# Autodesk Inventor assembly: NewChassis
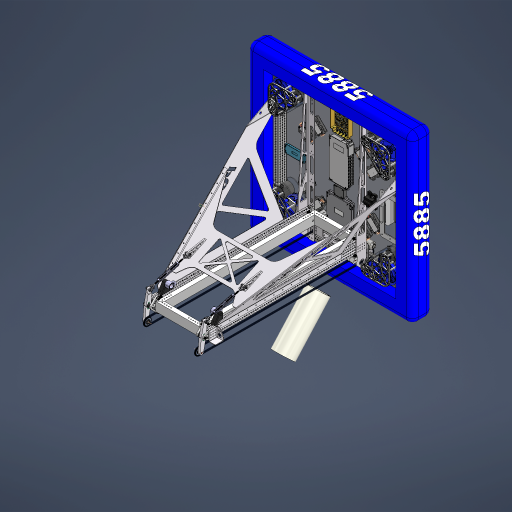
[picture p0: Inventor's stored thumbnail of the model, 512x512]
Saved by Autodesk Inventor 2024.3 (Build 283343000, 343)
## iProperties
ILogicPurgeVersion: 0.0.0.0
OnSaveVersion: 3.5.0.0
OnSaveAssembly: COREAutomationManager
Created: 2025-01-13
Part Number: NewChassis
Document SubType Name: Assembly
Designer: Marcus Tannini
Mfg Approved By: John.Thibert
Mass: 47914.5 g
Surface Area: 101218 cm^2
Volume: 49061.3 cm^3
Density: 0.976625 g/cm^3
ModelCat: Uncategorized
CN_MASS: 47.91
Author: Marcus Tannini
## Documents named in this file (44)
- \\clfs\homes\john.thibert\robot-test\#Poseidon 2025.iam
- \\clfs\homes\john.thibert\robot-test\ASSY,MK4i,Swerve_Module_INV.iam
- \\clfs\homes\john.thibert\robot-test\MAXTube-2x1-Holes.ipt
- \\clfs\homes\john.thibert\robot-test\BellyPanTop.ipt
- \\clfs\homes\john.thibert\robot-test\BellyPanBot.ipt
- \\clfs\homes\john.thibert\robot-test\BATTERY,12V.ipt
- \\clfs\homes\john.thibert\robot-test\CONTROLS,MAIN_BREAKER.ipt
- \\clfs\homes\john.thibert\robot-test\CONTROLS,MOTOR,NEO,550.ipt
- \\clfs\homes\john.thibert\robot-test\CONTROLS,PDH.ipt
- \\clfs\homes\john.thibert\robot-test\CONTROLS,PH.ipt
- \\clfs\homes\john.thibert\robot-test\CONTROLS,ROBO_RIO.ipt
- \\clfs\homes\john.thibert\robot-test\CONTROLS,SPARK_MAX.ipt
- \\clfs\homes\john.thibert\robot-test\CONTROLS,VRM.ipt
- \\clfs\homes\john.thibert\robot-test\COVER,SPARKMAX.ipt
- \\clfs\homes\john.thibert\robot-test\ModifiedCase(IncludesPatterning).iam
- \\clfs\homes\john.thibert\robot-test\PLATE,MOUNT,BATTERY,TOP.ipt
- \\clfs\homes\john.thibert\robot-test\PLATE,MOUNT,BATTERY,BOT.ipt
- \\clfs\homes\john.thibert\robot-test\MOUNT,STRAP,BATTERY.ipt
- \\clfs\homes\john.thibert\robot-test\SPACER,SPROCKET,IDLER,ELEVATOR.ipt
- \\clfs\homes\john.thibert\robot-test\22.ipt
- \\clfs\homes\john.thibert\robot-test\PLATE,MOUNT,DRIVE,ELEVATOR.ipt
- \\clfs\homes\john.thibert\robot-test\PLATE,BEARING,DRIVE,ELEVATOR.ipt
- \\clfs\homes\john.thibert\robot-test\PURCHASED,HEX_BEARING.ipt
- \\clfs\homes\john.thibert\robot-test\SHAFT,HEX,0.500in,DRIVE,ELEVATOR.ipt
- \\clfs\homes\john.thibert\robot-test\PLATE,SIDE,BRACE,RIGHT,ELEVATOR.ipt
- \\clfs\homes\john.thibert\robot-test\PLATE,SIDE,BRACE,LEFT,ELEVATOR.ipt
- \\clfs\homes\john.thibert\robot-test\PLATE,TURNBUCKLE,TENSIONER,CHAIN.ipt
- \\clfs\homes\john.thibert\robot-test\PLATE,BRACE,HORISONTAL,TOP,ELEVATOR.ipt
- \\clfs\homes\john.thibert\robot-test\TURNBUCKLE,0.25IN_CLEVIS.iam
- \\clfs\homes\john.thibert\robot-test\STAGE1,ELEVATOR.iam
- \\clfs\homes\john.thibert\robot-test\ASSY,MAIN,ELEVATOR.iam
- \\clfs\homes\john.thibert\robot-test\ANGLE,MOUNT,ELEVATOR.ipt
- \\clfs\homes\john.thibert\robot-test\ANGLE,MOUNT,ELEVATOR,MIRR.ipt
- \\clfs\homes\john.thibert\robot-test\FABRIC,BUMPERS.ipt
- \\clfs\homes\john.thibert\robot-test\9293K119_Constant-Force Spring.ipt
- \\clfs\homes\john.thibert\robot-test\MOUNT,SPRING,ELEVATOR.ipt
- \\clfs\homes\john.thibert\robot-test\MOUNT,SPRING,ELEVATOR,MIRR.ipt
- \\clfs\homes\john.thibert\robot-test\VersaPlanetary v2 Dual Stage 10_1 with RS 550 (1).iam
- \\clfs\homes\john.thibert\robot-test\60355K336_Ball Bearing.ipt
- \\clfs\homes\john.thibert\robot-test\91259A171_Alloy Steel Shoulder Screw.ipt
- \\clfs\homes\john.thibert\robot-test\BEARING,MOUNT,SIDE,ELEVATOR.ipt
- \\clfs\homes\john.thibert\robot-test\MOUNT,CABLE_TRACK,ELEVATOR.ipt
- \\clfs\homes\john.thibert\robot-test\CORAL.ipt
- \\clfs\homes\john.thibert\robot-test\BEARING,MOUNT,SIDE,ELEVATOR,MIRR.ipt
## Components (75 placed, 44 different names)
1. FABRIC,BUMPERS.ipt:1 — Flush:323, Mate:335, Mate:336
2. CORAL:1
3. BellyPanBot.ipt:1 — Mate:66, Mate:353, Mate:354
4. BellyPanTop.ipt:1 — Mate:62, Mate:63, Mate:65, Mate:70, Mate:71, Mate:82, Mate:84, Insert:7, Insert:8, Insert:9, Insert:10, Insert:11, Insert:12, Insert:13, Insert:14, Insert:15, Insert:16, Insert:17, Insert:18, Insert:19, Insert:20, Insert:21, Insert:22, Mate:111, Mate:113, Mate:114, Mate:116, Mate:117, Mate:118, Mate:119, Mate:121, Mate:122, Mate:123, Mate:124, Mate:125, Mate:126, Mate:127, Mate:130, Insert:23, Insert:24, Mate:223, Mate:308, Mate:320, Mate:349, Mate:350
5. MAXTube-2x1-Holes.ipt:1 — Mate:1, Mate:2, Mate:3, Mate:4, Mate:5, Mate:15, Mate:115, Mate:272
6. MAXTube-2x1-Holes.ipt:2 — Mate:6, Mate:7, Mate:8, Mate:9, Mate:10, Mate:11, Mate:62, Mate:309, Mate:310
7. MAXTube-2x1-Holes.ipt:3 — Mate:19, Mate:20, Mate:21, Mate:66, Mate:114, Mate:312, Mate:313, Mate:336
8. MAXTube-2x1-Holes.ipt:4 — Mate:12, Mate:13, Mate:14, Mate:16, Mate:17, Mate:18, Mate:29, Mate:63, Mate:271, Mate:353, Mate:354
9. MOUNT,STRAP,BATTERY.ipt:1 — Mate:357, Mate:358, Mate:359
10. PLATE,MOUNT,BATTERY,BOT.ipt:1 — Mate:320, Mate:321, Mate:351, Mate:352
11. PLATE,MOUNT,BATTERY,TOP.ipt:1 — Mate:127, Mate:349, Mate:350, Mate:351, Mate:352, Mate:356, Mate:357, Mate:358, Mate:359
12. BATTERY,12V.ipt:1 — Mate:321, Mate:356
13. CONTROLS,MAIN_BREAKER.ipt:1 — Mate:82, Mate:111, Mate:116
14. CONTROLS,MOTOR,NEO,550.ipt:1
15. CONTROLS,PDH.ipt:1 — Mate:113, Mate:117, Mate:118, Mate:119
16. CONTROLS,PH.ipt:1 — Insert:23, Insert:24
17. CONTROLS,ROBO_RIO.ipt:1 — Mate:124, Mate:125, Mate:126
18. CONTROLS,SPARK_MAX.ipt:1 — Mate:84, Mate:85, Mate:86, Mate:87
19. CONTROLS,VRM.ipt:1 — Mate:121, Mate:122, Mate:123
20. ModifiedCase(IncludesPatterning).iam:1 [sub-assembly] — Mate:130
21. 22.ipt:1 — Mate:227, Angle:6
22. 22.ipt:2 — Mate:233, Angle:4, Flush:14
23. 60355K336_Ball Bearing:1 — Mate:529, Mate:530, Mate:546
24. 60355K336_Ball Bearing:2 — Insert:51, Mate:545
25. 91259A171_Alloy Steel Shoulder Screw:1 — Mate:546
26. 91259A171_Alloy Steel Shoulder Screw:2 — Mate:545
27. 9293K119_Constant-Force Spring:1 — Mate:364, Mate:365
28. 9293K119_Constant-Force Spring:2 — Mate:370, Mate:371
29. ANGLE,MOUNT,ELEVATOR,MIRR.ipt:1 — Mate:308, Mate:309, Mate:310, Mate:311, Mate:312, Mate:313, Mate:314, Mate:315, Flush:329
30. ANGLE,MOUNT,ELEVATOR.ipt:1 — Mate:65, Mate:70, Mate:71, Mate:161, Mate:162, Mate:224, STAGE1 LOWER LIMIT, STAGE1 MIN
31. ASSY,MAIN,ELEVATOR.iam:1 [sub-assembly] — Mate:161, Mate:162, Flush:19, Mate:297, STAGE1 UPPER LIMIT, STAGE1 MAX, Mate:311, Mate:314, Mate:315, Mate:363, Mate:362, Mate:366, Mate:367, Mate:368, Mate:369, Mate:535, Mate:534, Mate:536
32. BEARING,MOUNT,SIDE,ELEVATOR,MIRR:1 — Mate:542, Mate:543, Mate:544, Insert:51
33. BEARING,MOUNT,SIDE,ELEVATOR:1 — Flush:330, Mate:528, Mate:529, Mate:530, Mate:531
34. CONTROLS,MOTOR,NEO,550:3
35. CONTROLS,MOTOR,NEO,550:4
36. MOUNT,CABLE_TRACK,ELEVATOR:1 — Mate:535, Mate:534, Mate:536
37. MOUNT,SPRING,ELEVATOR,MIRR:1 — Mate:367, Mate:368, Mate:369, Mate:370, Mate:371
38. MOUNT,SPRING,ELEVATOR:1 — Mate:363, Mate:362, Mate:364, Mate:365, Mate:366
39. PLATE,BEARING,DRIVE,ELEVATOR.ipt:1 — Mate:226, Mate:227, Mate:228, Mate:229, Insert:50
40. PLATE,BEARING,DRIVE,ELEVATOR.ipt:2 — Mate:230, Mate:231, Mate:232, Insert:49, Mate:233, Mate:234
41. PLATE,BRACE,HORISONTAL,TOP,ELEVATOR.ipt:1 — Mate:285, Mate:286, Mate:289, Mate:290, Mate:291, Mate:295, Mate:296
42. PLATE,MOUNT,DRIVE,ELEVATOR.ipt:1 — Mate:223, Mate:224, Mate:226, Mate:228, Mate:229, Mate:230, Mate:231, Mate:232, Flush:329, Mate:469, Mate:470, Mate:471, Mate:472, Mate:473, Mate:474
43. PLATE,SIDE,BRACE,LEFT,ELEVATOR.ipt:1 — Mate:271, Mate:289, Mate:290, Mate:291, Mate:335
44. PLATE,SIDE,BRACE,RIGHT,ELEVATOR.ipt:1 — Mate:272
45. PLATE,TURNBUCKLE,TENSIONER,CHAIN.ipt:1 — Mate:285, Mate:296
46. PLATE,TURNBUCKLE,TENSIONER,CHAIN.ipt:2 — Mate:286, Mate:295
47. PURCHASED,HEX_BEARING.ipt:1 — Insert:49, Angle:5
48. PURCHASED,HEX_BEARING.ipt:2 — Insert:50, Angle:7
49. SHAFT,HEX,0.500in,DRIVE,ELEVATOR.ipt:1 — Mate:234, Angle:4, Angle:5, Angle:6, Angle:7, Flush:14
50. SPACER,SPROCKET,IDLER,ELEVATOR.ipt:1
51. SPACER,SPROCKET,IDLER,ELEVATOR.ipt:2
52. STAGE1,ELEVATOR.iam:1 [sub-assembly] — Flush:19, Mate:297, STAGE1 LOWER LIMIT, STAGE1 UPPER LIMIT, STAGE1 MIN, STAGE1 MAX, Flush:330, Mate:528, Mate:531, Mate:542, Mate:543, Mate:544
53. TURNBUCKLE,0.25IN_CLEVIS.iam:1 [sub-assembly]
54. TURNBUCKLE,0.25IN_CLEVIS.iam:2 [sub-assembly]
55. VersaPlanetary v2 Dual Stage 10_1 with RS 550 (1):1 [sub-assembly] — Mate:472, Mate:473, Mate:474
56. VersaPlanetary v2 Dual Stage 10_1 with RS 550 (1):2 [sub-assembly] — Mate:469, Mate:470, Mate:471
57. ASSY,MK4i,Swerve_Module_INV.iam:1 [sub-assembly] — Mate:1, Mate:2, Mate:15
58. ASSY,MK4i,Swerve_Module_INV.iam:2 [sub-assembly] — Mate:3, Mate:4, Mate:5, Mate:6, Mate:7, Mate:8
59. ASSY,MK4i,Swerve_Module_INV.iam:3 [sub-assembly] — Mate:9, Mate:10, Mate:11, Mate:12, Mate:13, Mate:14
60. ASSY,MK4i,Swerve_Module_INV.iam:4 [sub-assembly] — Mate:16, Mate:17, Mate:18, Mate:19, Mate:20, Mate:21, Mate:67
61. CONTROLS,SPARK_MAX.ipt:2
62. CONTROLS,SPARK_MAX.ipt:3
63. CONTROLS,SPARK_MAX.ipt:4
64. CONTROLS,SPARK_MAX.ipt:5
65. CONTROLS,SPARK_MAX.ipt:6
66. CONTROLS,SPARK_MAX.ipt:7
67. CONTROLS,SPARK_MAX.ipt:8
68. COVER,SPARKMAX.ipt:1 — Mate:85, Mate:86, Mate:87, Insert:7, Insert:8
69. COVER,SPARKMAX.ipt:2 — Insert:9, Insert:10
70. COVER,SPARKMAX.ipt:3 — Insert:11, Insert:12
71. COVER,SPARKMAX.ipt:4 — Insert:13, Insert:14
72. COVER,SPARKMAX.ipt:5 — Insert:17, Insert:18
73. COVER,SPARKMAX.ipt:6 — Insert:15, Insert:16
74. COVER,SPARKMAX.ipt:7 — Insert:21, Insert:22
75. COVER,SPARKMAX.ipt:8 — Insert:19, Insert:20
## Relationships (203: Mate 167, Insert 25, Flush 7, Angle 4)
- Mate:1: MAXTube-2x1-Holes.ipt:1 ↔ ASSY,MK4i,Swerve_Module_INV.iam:1
- Mate:2: MAXTube-2x1-Holes.ipt:1 ↔ ASSY,MK4i,Swerve_Module_INV.iam:1
- Mate:3: MAXTube-2x1-Holes.ipt:1 ↔ ASSY,MK4i,Swerve_Module_INV.iam:2
- Mate:4: MAXTube-2x1-Holes.ipt:1 ↔ ASSY,MK4i,Swerve_Module_INV.iam:2
- Mate:5: MAXTube-2x1-Holes.ipt:1 ↔ ASSY,MK4i,Swerve_Module_INV.iam:2
- Mate:6: MAXTube-2x1-Holes.ipt:2 ↔ ASSY,MK4i,Swerve_Module_INV.iam:2
- Mate:7: MAXTube-2x1-Holes.ipt:2 ↔ ASSY,MK4i,Swerve_Module_INV.iam:2
- Mate:8: MAXTube-2x1-Holes.ipt:2 ↔ ASSY,MK4i,Swerve_Module_INV.iam:2
- Mate:9: MAXTube-2x1-Holes.ipt:2 ↔ ASSY,MK4i,Swerve_Module_INV.iam:3
- Mate:10: MAXTube-2x1-Holes.ipt:2 ↔ ASSY,MK4i,Swerve_Module_INV.iam:3
- Mate:11: MAXTube-2x1-Holes.ipt:2 ↔ ASSY,MK4i,Swerve_Module_INV.iam:3
- Mate:12: MAXTube-2x1-Holes.ipt:4 ↔ ASSY,MK4i,Swerve_Module_INV.iam:3
- Mate:13: MAXTube-2x1-Holes.ipt:4 ↔ ASSY,MK4i,Swerve_Module_INV.iam:3
- Mate:14: MAXTube-2x1-Holes.ipt:4 ↔ ASSY,MK4i,Swerve_Module_INV.iam:3
- Mate:15: MAXTube-2x1-Holes.ipt:1 ↔ ASSY,MK4i,Swerve_Module_INV.iam:1
- Mate:16: MAXTube-2x1-Holes.ipt:4 ↔ ASSY,MK4i,Swerve_Module_INV.iam:4
- Mate:17: MAXTube-2x1-Holes.ipt:4 ↔ ASSY,MK4i,Swerve_Module_INV.iam:4
- Mate:18: MAXTube-2x1-Holes.ipt:4 ↔ ASSY,MK4i,Swerve_Module_INV.iam:4
- Mate:19: MAXTube-2x1-Holes.ipt:3 ↔ ASSY,MK4i,Swerve_Module_INV.iam:4
- Mate:20: MAXTube-2x1-Holes.ipt:3 ↔ ASSY,MK4i,Swerve_Module_INV.iam:4
- Mate:21: MAXTube-2x1-Holes.ipt:3 ↔ ASSY,MK4i,Swerve_Module_INV.iam:4
- Mate:29 (-6.35 mm): MAXTube-2x1-Holes.ipt:4
- Mate:62: BellyPanTop.ipt:1 ↔ MAXTube-2x1-Holes.ipt:2
- Mate:63: BellyPanTop.ipt:1 ↔ MAXTube-2x1-Holes.ipt:4
- Mate:65: BellyPanTop.ipt:1 ↔ ANGLE,MOUNT,ELEVATOR.ipt:1
- Mate:66: BellyPanBot.ipt:1 ↔ MAXTube-2x1-Holes.ipt:3
- Mate:67 (35.56 mm): ASSY,MK4i,Swerve_Module_INV.iam:4
- Mate:70: BellyPanTop.ipt:1 ↔ ANGLE,MOUNT,ELEVATOR.ipt:1
- Mate:71: BellyPanTop.ipt:1 ↔ ANGLE,MOUNT,ELEVATOR.ipt:1
- Mate:321: PLATE,MOUNT,BATTERY,BOT.ipt:1 ↔ BATTERY,12V.ipt:1
- Mate:82: BellyPanTop.ipt:1 ↔ CONTROLS,MAIN_BREAKER.ipt:1
- Mate:84: BellyPanTop.ipt:1 ↔ CONTROLS,SPARK_MAX.ipt:1
- Mate:85: CONTROLS,SPARK_MAX.ipt:1 ↔ COVER,SPARKMAX.ipt:1
- Mate:86: CONTROLS,SPARK_MAX.ipt:1 ↔ COVER,SPARKMAX.ipt:1
- Mate:87: CONTROLS,SPARK_MAX.ipt:1 ↔ COVER,SPARKMAX.ipt:1
- Insert:7: BellyPanTop.ipt:1 ↔ COVER,SPARKMAX.ipt:1
- Insert:8: BellyPanTop.ipt:1 ↔ COVER,SPARKMAX.ipt:1
- [Mate]: CONTROLS,SPARK_MAX.ipt:2 ↔ COVER,SPARKMAX.ipt:2
- [Mate]: CONTROLS,SPARK_MAX.ipt:2 ↔ COVER,SPARKMAX.ipt:2
- [Mate]: CONTROLS,SPARK_MAX.ipt:2 ↔ COVER,SPARKMAX.ipt:2
- [Mate]: CONTROLS,SPARK_MAX.ipt:3 ↔ COVER,SPARKMAX.ipt:3
- [Mate]: CONTROLS,SPARK_MAX.ipt:3 ↔ COVER,SPARKMAX.ipt:3
- [Mate]: CONTROLS,SPARK_MAX.ipt:3 ↔ COVER,SPARKMAX.ipt:3
- [Mate]: CONTROLS,SPARK_MAX.ipt:4 ↔ COVER,SPARKMAX.ipt:4
- [Mate]: CONTROLS,SPARK_MAX.ipt:4 ↔ COVER,SPARKMAX.ipt:4
- [Mate]: CONTROLS,SPARK_MAX.ipt:4 ↔ COVER,SPARKMAX.ipt:4
- [Mate]: CONTROLS,SPARK_MAX.ipt:5 ↔ COVER,SPARKMAX.ipt:5
- [Mate]: CONTROLS,SPARK_MAX.ipt:5 ↔ COVER,SPARKMAX.ipt:5
- [Mate]: CONTROLS,SPARK_MAX.ipt:5 ↔ COVER,SPARKMAX.ipt:5
- [Mate]: CONTROLS,SPARK_MAX.ipt:6 ↔ COVER,SPARKMAX.ipt:6
- [Mate]: CONTROLS,SPARK_MAX.ipt:6 ↔ COVER,SPARKMAX.ipt:6
- [Mate]: CONTROLS,SPARK_MAX.ipt:6 ↔ COVER,SPARKMAX.ipt:6
- [Mate]: CONTROLS,SPARK_MAX.ipt:7 ↔ COVER,SPARKMAX.ipt:7
- [Mate]: CONTROLS,SPARK_MAX.ipt:7 ↔ COVER,SPARKMAX.ipt:7
- [Mate]: CONTROLS,SPARK_MAX.ipt:7 ↔ COVER,SPARKMAX.ipt:7
- [Mate]: CONTROLS,SPARK_MAX.ipt:8 ↔ COVER,SPARKMAX.ipt:8
- [Mate]: CONTROLS,SPARK_MAX.ipt:8 ↔ COVER,SPARKMAX.ipt:8
- [Mate]: CONTROLS,SPARK_MAX.ipt:8 ↔ COVER,SPARKMAX.ipt:8
- Insert:9: BellyPanTop.ipt:1 ↔ COVER,SPARKMAX.ipt:2
- Insert:10: BellyPanTop.ipt:1 ↔ COVER,SPARKMAX.ipt:2
- Insert:11: BellyPanTop.ipt:1 ↔ COVER,SPARKMAX.ipt:3
- Insert:12: BellyPanTop.ipt:1 ↔ COVER,SPARKMAX.ipt:3
- Insert:13: BellyPanTop.ipt:1 ↔ COVER,SPARKMAX.ipt:4
- Insert:14: BellyPanTop.ipt:1 ↔ COVER,SPARKMAX.ipt:4
- Insert:15: BellyPanTop.ipt:1 ↔ COVER,SPARKMAX.ipt:6
- Insert:16: BellyPanTop.ipt:1 ↔ COVER,SPARKMAX.ipt:6
- Insert:17: BellyPanTop.ipt:1 ↔ COVER,SPARKMAX.ipt:5
- Insert:18: BellyPanTop.ipt:1 ↔ COVER,SPARKMAX.ipt:5
- Insert:19: BellyPanTop.ipt:1 ↔ COVER,SPARKMAX.ipt:8
- Insert:20: BellyPanTop.ipt:1 ↔ COVER,SPARKMAX.ipt:8
- Insert:21: BellyPanTop.ipt:1 ↔ COVER,SPARKMAX.ipt:7
- Insert:22: BellyPanTop.ipt:1 ↔ COVER,SPARKMAX.ipt:7
- Mate:111: BellyPanTop.ipt:1 ↔ CONTROLS,MAIN_BREAKER.ipt:1
- Mate:113: BellyPanTop.ipt:1 ↔ CONTROLS,PDH.ipt:1
- Mate:114: BellyPanTop.ipt:1 ↔ MAXTube-2x1-Holes.ipt:3
- Mate:115 (-374.65 mm): MAXTube-2x1-Holes.ipt:1
- Mate:116 (0.254 mm): BellyPanTop.ipt:1 ↔ CONTROLS,MAIN_BREAKER.ipt:1
- Mate:117: BellyPanTop.ipt:1 ↔ CONTROLS,PDH.ipt:1
- Mate:118: BellyPanTop.ipt:1 ↔ CONTROLS,PDH.ipt:1
- Mate:119: BellyPanTop.ipt:1 ↔ CONTROLS,PDH.ipt:1
- Mate:121: BellyPanTop.ipt:1 ↔ CONTROLS,VRM.ipt:1
- Mate:122: BellyPanTop.ipt:1 ↔ CONTROLS,VRM.ipt:1
- Mate:123: BellyPanTop.ipt:1 ↔ CONTROLS,VRM.ipt:1
- Mate:124: BellyPanTop.ipt:1 ↔ CONTROLS,ROBO_RIO.ipt:1
- Mate:125: BellyPanTop.ipt:1 ↔ CONTROLS,ROBO_RIO.ipt:1
- Mate:126: BellyPanTop.ipt:1 ↔ CONTROLS,ROBO_RIO.ipt:1
- Mate:127: BellyPanTop.ipt:1 ↔ PLATE,MOUNT,BATTERY,TOP.ipt:1
- Mate:130: BellyPanTop.ipt:1 ↔ ModifiedCase(IncludesPatterning).iam:1
- Insert:23: BellyPanTop.ipt:1 ↔ CONTROLS,PH.ipt:1
- Insert:24: BellyPanTop.ipt:1 ↔ CONTROLS,PH.ipt:1
- Mate:161: ANGLE,MOUNT,ELEVATOR.ipt:1 ↔ ASSY,MAIN,ELEVATOR.iam:1
- Mate:162: ANGLE,MOUNT,ELEVATOR.ipt:1 ↔ ASSY,MAIN,ELEVATOR.iam:1
- [Mate]: ANGLE,MOUNT,ELEVATOR.ipt:1 ↔ ASSY,MAIN,ELEVATOR.iam:1
- [Insert]: ASSY,MAIN,ELEVATOR.iam:1 ↔ SPACER,SPROCKET,IDLER,ELEVATOR.ipt:1
- [Insert]: ASSY,MAIN,ELEVATOR.iam:1 ↔ SPACER,SPROCKET,IDLER,ELEVATOR.ipt:1
- [Flush]: 22.ipt:1 ↔ ASSY,MAIN,ELEVATOR.iam:1
- [Insert]: ASSY,MAIN,ELEVATOR.iam:1 ↔ SPACER,SPROCKET,IDLER,ELEVATOR.ipt:2
- [Insert]: ASSY,MAIN,ELEVATOR.iam:1 ↔ SPACER,SPROCKET,IDLER,ELEVATOR.ipt:2
- Mate:223: BellyPanTop.ipt:1 ↔ PLATE,MOUNT,DRIVE,ELEVATOR.ipt:1
- Mate:224: ANGLE,MOUNT,ELEVATOR.ipt:1 ↔ PLATE,MOUNT,DRIVE,ELEVATOR.ipt:1
- Mate:226: PLATE,BEARING,DRIVE,ELEVATOR.ipt:1 ↔ PLATE,MOUNT,DRIVE,ELEVATOR.ipt:1
- Mate:227: 22.ipt:1 ↔ PLATE,BEARING,DRIVE,ELEVATOR.ipt:1
- Mate:228: PLATE,BEARING,DRIVE,ELEVATOR.ipt:1 ↔ PLATE,MOUNT,DRIVE,ELEVATOR.ipt:1
- Mate:229: PLATE,BEARING,DRIVE,ELEVATOR.ipt:1 ↔ PLATE,MOUNT,DRIVE,ELEVATOR.ipt:1
- Mate:230: PLATE,BEARING,DRIVE,ELEVATOR.ipt:2 ↔ PLATE,MOUNT,DRIVE,ELEVATOR.ipt:1
- Mate:231: PLATE,BEARING,DRIVE,ELEVATOR.ipt:2 ↔ PLATE,MOUNT,DRIVE,ELEVATOR.ipt:1
- Mate:232: PLATE,BEARING,DRIVE,ELEVATOR.ipt:2 ↔ PLATE,MOUNT,DRIVE,ELEVATOR.ipt:1
- Insert:49: PLATE,BEARING,DRIVE,ELEVATOR.ipt:2 ↔ PURCHASED,HEX_BEARING.ipt:1
- Insert:50: PLATE,BEARING,DRIVE,ELEVATOR.ipt:1 ↔ PURCHASED,HEX_BEARING.ipt:2
- Mate:233: 22.ipt:2 ↔ PLATE,BEARING,DRIVE,ELEVATOR.ipt:2
- Mate:234: PLATE,BEARING,DRIVE,ELEVATOR.ipt:2 ↔ SHAFT,HEX,0.500in,DRIVE,ELEVATOR.ipt:1
- Angle:4 (0 deg): 22.ipt:2 ↔ SHAFT,HEX,0.500in,DRIVE,ELEVATOR.ipt:1
- Angle:5 (0 deg): PURCHASED,HEX_BEARING.ipt:1 ↔ SHAFT,HEX,0.500in,DRIVE,ELEVATOR.ipt:1
- Angle:6 (0 deg): 22.ipt:1 ↔ SHAFT,HEX,0.500in,DRIVE,ELEVATOR.ipt:1
- Angle:7 (0 deg): PURCHASED,HEX_BEARING.ipt:2 ↔ SHAFT,HEX,0.500in,DRIVE,ELEVATOR.ipt:1
- [Flush]: 22.ipt:2 ↔ ASSY,MAIN,ELEVATOR.iam:1
- [Mate]: ASSY,MAIN,ELEVATOR.iam:1 ↔ PLATE,SIDE,BRACE,LEFT,ELEVATOR.ipt:1
- [Mate]: ASSY,MAIN,ELEVATOR.iam:1 ↔ PLATE,SIDE,BRACE,LEFT,ELEVATOR.ipt:1
- [Mate]: 22.ipt:1 ↔ ASSY,MAIN,ELEVATOR.iam:1
- Flush:14 (-15.875 mm): 22.ipt:2 ↔ SHAFT,HEX,0.500in,DRIVE,ELEVATOR.ipt:1
- [Mate]: ASSY,MAIN,ELEVATOR.iam:1 ↔ PLATE,SIDE,BRACE,LEFT,ELEVATOR.ipt:1
- [Mate]: ASSY,MAIN,ELEVATOR.iam:1 ↔ PLATE,SIDE,BRACE,RIGHT,ELEVATOR.ipt:1
- [Mate]: ASSY,MAIN,ELEVATOR.iam:1 ↔ PLATE,SIDE,BRACE,RIGHT,ELEVATOR.ipt:1
- [Mate]: ASSY,MAIN,ELEVATOR.iam:1 ↔ PLATE,SIDE,BRACE,RIGHT,ELEVATOR.ipt:1
- Mate:271: MAXTube-2x1-Holes.ipt:4 ↔ PLATE,SIDE,BRACE,LEFT,ELEVATOR.ipt:1
- Mate:272: MAXTube-2x1-Holes.ipt:1 ↔ PLATE,SIDE,BRACE,RIGHT,ELEVATOR.ipt:1
- [Mate]: ASSY,MAIN,ELEVATOR.iam:1 ↔ TURNBUCKLE,0.25IN_CLEVIS.iam:1
- [Mate]: ASSY,MAIN,ELEVATOR.iam:1 ↔ TURNBUCKLE,0.25IN_CLEVIS.iam:1
- [Mate]: ASSY,MAIN,ELEVATOR.iam:1 ↔ TURNBUCKLE,0.25IN_CLEVIS.iam:2
- [Mate]: ASSY,MAIN,ELEVATOR.iam:1 ↔ TURNBUCKLE,0.25IN_CLEVIS.iam:2
- Mate:285: PLATE,BRACE,HORISONTAL,TOP,ELEVATOR.ipt:1 ↔ PLATE,TURNBUCKLE,TENSIONER,CHAIN.ipt:1
- Mate:286: PLATE,BRACE,HORISONTAL,TOP,ELEVATOR.ipt:1 ↔ PLATE,TURNBUCKLE,TENSIONER,CHAIN.ipt:2
- Mate:289: PLATE,BRACE,HORISONTAL,TOP,ELEVATOR.ipt:1 ↔ PLATE,SIDE,BRACE,LEFT,ELEVATOR.ipt:1
- Mate:290: PLATE,BRACE,HORISONTAL,TOP,ELEVATOR.ipt:1 ↔ PLATE,SIDE,BRACE,LEFT,ELEVATOR.ipt:1
- Mate:291: PLATE,BRACE,HORISONTAL,TOP,ELEVATOR.ipt:1 ↔ PLATE,SIDE,BRACE,LEFT,ELEVATOR.ipt:1
- [Mate]: 22.ipt:2 ↔ ASSY,MAIN,ELEVATOR.iam:1
- Mate:295: PLATE,BRACE,HORISONTAL,TOP,ELEVATOR.ipt:1 ↔ PLATE,TURNBUCKLE,TENSIONER,CHAIN.ipt:2
- Mate:296: PLATE,BRACE,HORISONTAL,TOP,ELEVATOR.ipt:1 ↔ PLATE,TURNBUCKLE,TENSIONER,CHAIN.ipt:1
- Flush:19: ASSY,MAIN,ELEVATOR.iam:1 ↔ STAGE1,ELEVATOR.iam:1
- Mate:297: ASSY,MAIN,ELEVATOR.iam:1 ↔ STAGE1,ELEVATOR.iam:1
- STAGE1 LOWER LIMIT [Mate]: ANGLE,MOUNT,ELEVATOR.ipt:1 ↔ STAGE1,ELEVATOR.iam:1
- STAGE1 UPPER LIMIT [Mate]: ASSY,MAIN,ELEVATOR.iam:1 ↔ STAGE1,ELEVATOR.iam:1
- STAGE1 MIN [Mate]: ANGLE,MOUNT,ELEVATOR.ipt:1 ↔ STAGE1,ELEVATOR.iam:1
- STAGE1 MAX [Mate] (3.175 mm): ASSY,MAIN,ELEVATOR.iam:1 ↔ STAGE1,ELEVATOR.iam:1
- Mate:308: BellyPanTop.ipt:1 ↔ ANGLE,MOUNT,ELEVATOR,MIRR.ipt:1
- Mate:309: MAXTube-2x1-Holes.ipt:2 ↔ ANGLE,MOUNT,ELEVATOR,MIRR.ipt:1
- Mate:310: MAXTube-2x1-Holes.ipt:2 ↔ ANGLE,MOUNT,ELEVATOR,MIRR.ipt:1
- Mate:311: ANGLE,MOUNT,ELEVATOR,MIRR.ipt:1 ↔ ASSY,MAIN,ELEVATOR.iam:1
- Mate:312: MAXTube-2x1-Holes.ipt:3 ↔ ANGLE,MOUNT,ELEVATOR,MIRR.ipt:1
- Mate:313: MAXTube-2x1-Holes.ipt:3 ↔ ANGLE,MOUNT,ELEVATOR,MIRR.ipt:1
- Mate:314: ANGLE,MOUNT,ELEVATOR,MIRR.ipt:1 ↔ ASSY,MAIN,ELEVATOR.iam:1
- Mate:315: ANGLE,MOUNT,ELEVATOR,MIRR.ipt:1 ↔ ASSY,MAIN,ELEVATOR.iam:1
- Mate:320: BellyPanTop.ipt:1 ↔ PLATE,MOUNT,BATTERY,BOT.ipt:1
- Flush:323 (146.05 mm): FABRIC,BUMPERS.ipt:1
- Mate:335 (3.175 mm): FABRIC,BUMPERS.ipt:1 ↔ PLATE,SIDE,BRACE,LEFT,ELEVATOR.ipt:1
- Mate:336 (6.35 mm): FABRIC,BUMPERS.ipt:1 ↔ MAXTube-2x1-Holes.ipt:3
- Mate:349: BellyPanTop.ipt:1 ↔ PLATE,MOUNT,BATTERY,TOP.ipt:1
- Mate:350: BellyPanTop.ipt:1 ↔ PLATE,MOUNT,BATTERY,TOP.ipt:1
- Mate:351: PLATE,MOUNT,BATTERY,BOT.ipt:1 ↔ PLATE,MOUNT,BATTERY,TOP.ipt:1
- Mate:352: PLATE,MOUNT,BATTERY,BOT.ipt:1 ↔ PLATE,MOUNT,BATTERY,TOP.ipt:1
- Mate:353: BellyPanBot.ipt:1 ↔ MAXTube-2x1-Holes.ipt:4
- Mate:354: BellyPanBot.ipt:1 ↔ MAXTube-2x1-Holes.ipt:4
- Mate:356 (19.05 mm): PLATE,MOUNT,BATTERY,TOP.ipt:1 ↔ BATTERY,12V.ipt:1
- Mate:357: MOUNT,STRAP,BATTERY.ipt:1 ↔ PLATE,MOUNT,BATTERY,TOP.ipt:1
- Mate:358: MOUNT,STRAP,BATTERY.ipt:1 ↔ PLATE,MOUNT,BATTERY,TOP.ipt:1
- Mate:359: MOUNT,STRAP,BATTERY.ipt:1 ↔ PLATE,MOUNT,BATTERY,TOP.ipt:1
- Mate:363: ASSY,MAIN,ELEVATOR.iam:1 ↔ MOUNT,SPRING,ELEVATOR:1
- Mate:362: ASSY,MAIN,ELEVATOR.iam:1 ↔ MOUNT,SPRING,ELEVATOR:1
- Mate:364: 9293K119_Constant-Force Spring:1 ↔ MOUNT,SPRING,ELEVATOR:1
- Mate:365 (1.5875 mm): 9293K119_Constant-Force Spring:1 ↔ MOUNT,SPRING,ELEVATOR:1
- Mate:366: ASSY,MAIN,ELEVATOR.iam:1 ↔ MOUNT,SPRING,ELEVATOR:1
- Mate:367: ASSY,MAIN,ELEVATOR.iam:1 ↔ MOUNT,SPRING,ELEVATOR,MIRR:1
- Mate:368: ASSY,MAIN,ELEVATOR.iam:1 ↔ MOUNT,SPRING,ELEVATOR,MIRR:1
- Mate:369: ASSY,MAIN,ELEVATOR.iam:1 ↔ MOUNT,SPRING,ELEVATOR,MIRR:1
- Mate:370: 9293K119_Constant-Force Spring:2 ↔ MOUNT,SPRING,ELEVATOR,MIRR:1
- Mate:371 (1.5875 mm): 9293K119_Constant-Force Spring:2 ↔ MOUNT,SPRING,ELEVATOR,MIRR:1
- Flush:329: ANGLE,MOUNT,ELEVATOR,MIRR.ipt:1 ↔ PLATE,MOUNT,DRIVE,ELEVATOR.ipt:1
- [Mate]: CONTROLS,MOTOR,NEO,550:3 ↔ VersaPlanetary v2 Dual Stage 10_1 with RS 550 (1):1
- [Mate]: CONTROLS,MOTOR,NEO,550:3 ↔ VersaPlanetary v2 Dual Stage 10_1 with RS 550 (1):1
- [Mate]: CONTROLS,MOTOR,NEO,550:4 ↔ VersaPlanetary v2 Dual Stage 10_1 with RS 550 (1):2
- [Mate]: CONTROLS,MOTOR,NEO,550:4 ↔ VersaPlanetary v2 Dual Stage 10_1 with RS 550 (1):2
- Mate:469: PLATE,MOUNT,DRIVE,ELEVATOR.ipt:1 ↔ VersaPlanetary v2 Dual Stage 10_1 with RS 550 (1):2
- Mate:470: PLATE,MOUNT,DRIVE,ELEVATOR.ipt:1 ↔ VersaPlanetary v2 Dual Stage 10_1 with RS 550 (1):2
- Mate:471: PLATE,MOUNT,DRIVE,ELEVATOR.ipt:1 ↔ VersaPlanetary v2 Dual Stage 10_1 with RS 550 (1):2
- Mate:472: PLATE,MOUNT,DRIVE,ELEVATOR.ipt:1 ↔ VersaPlanetary v2 Dual Stage 10_1 with RS 550 (1):1
- Mate:473: PLATE,MOUNT,DRIVE,ELEVATOR.ipt:1 ↔ VersaPlanetary v2 Dual Stage 10_1 with RS 550 (1):1
- Mate:474: PLATE,MOUNT,DRIVE,ELEVATOR.ipt:1 ↔ VersaPlanetary v2 Dual Stage 10_1 with RS 550 (1):1
- [Mate]: 60355K336_Ball Bearing:1 ↔ 91259A171_Alloy Steel Shoulder Screw:1
- Flush:330: BEARING,MOUNT,SIDE,ELEVATOR:1 ↔ STAGE1,ELEVATOR.iam:1
- Mate:528: BEARING,MOUNT,SIDE,ELEVATOR:1 ↔ STAGE1,ELEVATOR.iam:1
- Mate:529: 60355K336_Ball Bearing:1 ↔ BEARING,MOUNT,SIDE,ELEVATOR:1
- Mate:530: 60355K336_Ball Bearing:1 ↔ BEARING,MOUNT,SIDE,ELEVATOR:1
- Mate:531: BEARING,MOUNT,SIDE,ELEVATOR:1 ↔ STAGE1,ELEVATOR.iam:1
- Mate:535: ASSY,MAIN,ELEVATOR.iam:1 ↔ MOUNT,CABLE_TRACK,ELEVATOR:1
- Mate:534: ASSY,MAIN,ELEVATOR.iam:1 ↔ MOUNT,CABLE_TRACK,ELEVATOR:1
- Mate:536: ASSY,MAIN,ELEVATOR.iam:1 ↔ MOUNT,CABLE_TRACK,ELEVATOR:1
- [Mate]: 60355K336_Ball Bearing:2 ↔ 91259A171_Alloy Steel Shoulder Screw:2
- Mate:542: BEARING,MOUNT,SIDE,ELEVATOR,MIRR:1 ↔ STAGE1,ELEVATOR.iam:1
- Mate:543: BEARING,MOUNT,SIDE,ELEVATOR,MIRR:1 ↔ STAGE1,ELEVATOR.iam:1
- Mate:544: BEARING,MOUNT,SIDE,ELEVATOR,MIRR:1 ↔ STAGE1,ELEVATOR.iam:1
- Insert:51: 60355K336_Ball Bearing:2 ↔ BEARING,MOUNT,SIDE,ELEVATOR,MIRR:1
- Mate:545: 60355K336_Ball Bearing:2 ↔ 91259A171_Alloy Steel Shoulder Screw:2
- Mate:546: 60355K336_Ball Bearing:1 ↔ 91259A171_Alloy Steel Shoulder Screw:1
## Named parameters: d160_d155 = 0 mm, d161_d156 = 0 mm, d162_d157 = 0 mm, d163_d155 = 0 mm, d164_d156 = 0 mm, d165_d157 = 0 mm, d166_d155 = 0 mm, d167_d156 = 0 mm, d168_d157 = 0 mm, d169_d155 = 0 mm, d170_d156 = 0 mm, d171_d157 = 0 mm, d172_d155 = 0 mm, d173_d156 = 0 mm, d174_d157 = 0 mm, d175_d155 = 0 mm, d176_d156 = 0 mm, d177_d157 = 0 mm, d178_d155 = 0 mm, d179_d156 = 0 mm, d180_d157 = 0 mm, d518_d513 = 0 mm, d875_d873 = 0 mm, d876_d874 = 0 mm, d967_d875_d873 = 0 mm, d968_d876_d874 = 0 mm, d1097_d52 = 0 mm
